# Autodesk Inventor assembly: force_sensor_v2
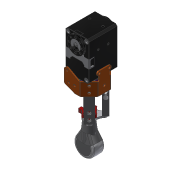
[picture p0: Inventor's stored thumbnail of the model, 180x180]
Saved by Autodesk Inventor 2019.4 (Build 234330000, 330)
## iProperties
Created: 2018-02-01
Part Number: force_sensor_v2
Material: 一般
Document SubType Name: Assembly
Designer: y6tada
Mass: 71.8116 g
Surface Area: 307.312 cm^2
Volume: 59.3643 cm^3
Density: 1.20968 g/cm^3
Author: y6tada
## Documents named in this file (18)
- C:\Workspace\Yunit8-HaptHexa\Hardware\Inventor\Tibia\_Tibia.iam
- C:\Workspace\Yunit8-HaptHexa\Hardware\Inventor\Tibia\leg_pipe_cfrp.ipt
- C:\Workspace\Yunit8-HaptHexa\Hardware\Inventor\X430\XL-430.iam
- C:\Workspace\Yunit8-HaptHexa\Hardware\Inventor\Tibia\plate.ipt
- C:\Workspace\Yunit8-HaptHexa\Hardware\Inventor\Tibia\load_cell_v2.ipt
- C:\Workspace\Yunit8-HaptHexa\Hardware\Inventor\Tibia\lod_holder.ipt
- C:\Workspace\Yunit8-HaptHexa\Hardware\Inventor\Tibia\con_sensor_lod.ipt
- C:\Workspace\Yunit8-HaptHexa\Hardware\Inventor\Tibia\z_sensor_base.ipt
- C:\Workspace\Yunit8-HaptHexa\Hardware\Inventor\Tibia\lod_base.ipt
- C:\Workspace\Yunit8-HaptHexa\Hardware\Inventor\Tibia\pin_2x15.ipt
- C:\Workspace\Yunit8-HaptHexa\Hardware\Inventor\Tibia\force_sensor_pcb_assy.iam
- C:\Workspace\GRIP_BASE_ASM.iam
- D:\2019.3 - HaptHexa\Hardware\Mech\Inventor\Tibia\_Tibia\AIP\FEA\csifsck2o.fins
- D:\2019.3 - HaptHexa\Hardware\Mech\Inventor\Tibia\_Tibia\AIP\FEA\csifsck2o.fsat
- D:\2019.3 - HaptHexa\Hardware\Mech\Inventor\Tibia\_Tibia\AIP\FEA\csifsck2o.ftes
- D:\2019.3 - HaptHexa\Hardware\Mech\Inventor\Tibia\_Tibia\AIP\FEA\csifsck2o.fwiz
- D:\2019.3 - HaptHexa\Hardware\Mech\Inventor\Tibia\_Tibia\AIP\FEA\csifsck9s.fmsh
- D:\2019.3 - HaptHexa\Hardware\Mech\Inventor\Tibia\_Tibia\AIP\FEA\csifsck9t.fres
## Components (13 placed, 11 different names)
1. XL-430:1 [sub-assembly] — メイト:29, メイト:30, メイト:31, フラッシュ:3, メイト:43
2. leg_pipe_cfrp:1 — メイト:40, メイト:41, メイト:46, メイト:47, メイト:52, メイト:59
3. plate:1 — メイト:29, メイト:30, メイト:31, メイト:34, メイト:35, メイト:36, メイト:37, メイト:38, メイト:39, 角度:2, メイト:48, メイト:49
4. load_cell_v2:1 — メイト:34, メイト:35, メイト:36, フラッシュ:1, メイト:55, フラッシュ:4
5. load_cell_v2:2 — メイト:37, メイト:38, メイト:39, メイト:56, フラッシュ:5
6. lod_holder:1 — メイト:40, 角度:2, フラッシュ:1, フラッシュ:2, メイト:42
7. con_sensor_lod:1 — フラッシュ:2, メイト:41, メイト:42
8. z_sensor_base:1 — メイト:43, メイト:48, メイト:49, メイト:50, メイト:51, メイト:53, メイト:57, メイト:58, 角度:3
9. lod_base:1 — メイト:46, メイト:47, メイト:50, メイト:51, メイト:53
10. pin_2x15:1 — メイト:55, フラッシュ:4
11. pin_2x15:2 — メイト:56, フラッシュ:5
12. force_sensor_pcb_assy:1 [sub-assembly] — メイト:57, メイト:58, 角度:3
13. GRIP_BASE_ASM:1 [sub-assembly] — メイト:59, フラッシュ:7
## Relationships (35: Mate 26, Flush 7, Angle 2)
- メイト:29 [Mate]: XL-430:1 ↔ plate:1
- メイト:30 [Mate]: XL-430:1 ↔ plate:1
- メイト:31 [Mate]: XL-430:1 ↔ plate:1
- メイト:34 [Mate]: plate:1 ↔ load_cell_v2:1
- メイト:35 [Mate]: plate:1 ↔ load_cell_v2:1
- メイト:36 [Mate]: plate:1 ↔ load_cell_v2:1
- メイト:37 [Mate]: plate:1 ↔ load_cell_v2:2
- メイト:38 [Mate]: plate:1 ↔ load_cell_v2:2
- メイト:39 [Mate]: plate:1 ↔ load_cell_v2:2
- メイト:40 [Mate]: leg_pipe_cfrp:1 ↔ lod_holder:1
- 角度:2 [Angle] (0 deg): plate:1 ↔ lod_holder:1
- フラッシュ:1 [Flush] (-1 mm): load_cell_v2:1 ↔ lod_holder:1
- フラッシュ:2 [Flush]: lod_holder:1 ↔ con_sensor_lod:1
- メイト:41 [Mate]: leg_pipe_cfrp:1 ↔ con_sensor_lod:1
- メイト:42 [Mate]: lod_holder:1 ↔ con_sensor_lod:1
- フラッシュ:3 [Flush] (3 mm): XL-430:1
- メイト:43 [Mate] (3 mm): XL-430:1 ↔ z_sensor_base:1
- メイト:46 [Mate]: leg_pipe_cfrp:1 ↔ lod_base:1
- メイト:47 [Mate]: leg_pipe_cfrp:1 ↔ lod_base:1
- メイト:48 [Mate]: plate:1 ↔ z_sensor_base:1
- メイト:49 [Mate]: plate:1 ↔ z_sensor_base:1
- メイト:50 [Mate]: z_sensor_base:1 ↔ lod_base:1
- メイト:51 [Mate]: z_sensor_base:1 ↔ lod_base:1
- メイト:52 [Mate]: leg_pipe_cfrp:1
- メイト:53 [Mate]: z_sensor_base:1 ↔ lod_base:1
- メイト:55 [Mate]: load_cell_v2:1 ↔ pin_2x15:1
- フラッシュ:4 [Flush] (3 mm): load_cell_v2:1 ↔ pin_2x15:1
- メイト:56 [Mate]: load_cell_v2:2 ↔ pin_2x15:2
- フラッシュ:5 [Flush] (3 mm): load_cell_v2:2 ↔ pin_2x15:2
- メイト:57 [Mate]: z_sensor_base:1 ↔ force_sensor_pcb_assy:1
- メイト:58 [Mate]: z_sensor_base:1 ↔ force_sensor_pcb_assy:1
- 角度:3 [Angle] (0 deg): z_sensor_base:1 ↔ force_sensor_pcb_assy:1
- フラッシュ:6 [Flush] (-125 mm)
- メイト:59 [Mate]: leg_pipe_cfrp:1 ↔ GRIP_BASE_ASM:1
- フラッシュ:7 [Flush] (12.2 mm): GRIP_BASE_ASM:1
## Named parameters: sa_0 = 1e-13, sa_1 = -6e-13, sa_2 = -500, sa_3 = -353.553, sa_4 = -5e-13, sa_5 = -353.553, sa_6 = -500, sa_7 = -0, sa_8 = -1e-13, sa_9 = -0, sa_10 = 500, sa_11 = -6e-13
note: some values were not read from the file. Shown as the stored number, unit unknown: "sa_0", "sa_1", "sa_2", "sa_3", "sa_4", "sa_5", "sa_6", "sa_7", "sa_8", "sa_9", "sa_10", "sa_11".
